# Autodesk Inventor assembly: KeyerFrontIambic
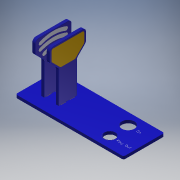
[picture p0: Inventor's stored thumbnail of the model, 180x180]
Saved by Autodesk Inventor 2016 (Build 200138000, 138)
## iProperties
Created: 2016-06-11
Part Number: KeyerFrontIambic
Document SubType Name: Assembly
Designer: Tyler
Author: Tyler
## Documents named in this file (3)
- C:\Users\Tyler\Documents\Small Projects\Personal\morse-practice-oscillator\Mechanicial\Key\KeyerFrontIambic.iam
- C:\Users\Tyler\Documents\Small Projects\Personal\morse-practice-oscillator\Mechanicial\Key\KeyerFront_Iambic.ipt
- C:\Users\Tyler\Documents\Small Projects\Personal\morse-practice-oscillator\Mechanicial\Key\KeyerPaddle.ipt
## Components (3 placed, 2 different names)
1. KeyerFront_Iambic:1 — Mate:1, Mate:2, Mate:3, Mate:6, Mate:7, Mate:8
2. KeyerPaddle:1 — Mate:6, Mate:7, Mate:8
3. KeyerPaddle:2 — Mate:1, Mate:2, Mate:3
## Relationships (6: Mate 6)
- Mate:1 (0.1 mm): KeyerFront_Iambic:1 ↔ KeyerPaddle:2
- Mate:2 (0.1 mm): KeyerFront_Iambic:1 ↔ KeyerPaddle:2
- Mate:3: KeyerFront_Iambic:1 ↔ KeyerPaddle:2
- Mate:6: KeyerFront_Iambic:1 ↔ KeyerPaddle:1
- Mate:7 (0.1 mm): KeyerFront_Iambic:1 ↔ KeyerPaddle:1
- Mate:8 (0.1 mm): KeyerFront_Iambic:1 ↔ KeyerPaddle:1
